# Autodesk Inventor assembly: Assembly X-Quad
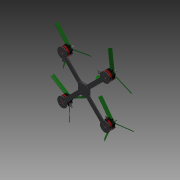
[picture p0: Inventor's stored thumbnail of the model, 180x180]
Saved by Autodesk Inventor 2015 (Build 190159000, 159)
## iProperties
Created: 2016-11-27
Part Number: Assembly X-Quad
Document SubType Name: Assembly
Designer: Hampus
Author: Hampus
## Documents named in this file (6)
- C:\Users\Hampus.Hampus-Dator\Desktop\Gymnasiearbete\Assembly X-Quad.iam
- C:\Users\Hampus.Hampus-Dator\Desktop\Gymnasiearbete\top.ipt
- C:\Users\Hampus.Hampus-Dator\Desktop\Gymnasiearbete\arm.ipt
- C:\Users\Hampus.Hampus-Dator\Desktop\Gymnasiearbete\botten.ipt
- D:\CAD3\Emax RS2205.ipt
- C:\Users\Hampus.Hampus-Dator\Desktop\Gymnasiearbete\DAL T5040.ipt
## Components (14 placed, 5 different names)
1. top:1 — Cylindrical:1, Rigid:1, Rigid:2, Cylindrical:2, Rotational:1
2. arm:1 — Rigid:2, Rotational:4
3. arm:2 — Cylindrical:1, Rotational:3
4. arm:3 — Cylindrical:2, Rotational:2
5. arm:4 — Rigid:1, Rigid:3
6. botten:1 — Rotational:1
7. Emax RS2205:1 — Rotational:4, Rigid:5
8. Emax RS2205:2 — Rigid:3, Rigid:4
9. Emax RS2205:3 — Rotational:3, Rigid:7
10. Emax RS2205:4 — Rotational:2, Rigid:6
11. DAL T5040:1 — Rigid:7
12. DAL T5040:2 — Rigid:6
13. DAL T5040:3 — Rigid:5
14. DAL T5040:4 — Rigid:4
## Relationships (13: WeldJoint 7, RevoluteJoint 4, CylindricalJoint 2)
- Cylindrical:1: top:1 ↔ arm:2
- Rigid:1 [WeldJoint]: top:1 ↔ arm:4
- Rigid:2 [WeldJoint]: top:1 ↔ arm:1
- Cylindrical:2: top:1 ↔ arm:3
- Rotational:1 [RevoluteJoint]: top:1 ↔ botten:1
- Rotational:2 [RevoluteJoint]: arm:3 ↔ Emax RS2205:4
- Rotational:3 [RevoluteJoint]: arm:2 ↔ Emax RS2205:3
- Rigid:3 [WeldJoint]: arm:4 ↔ Emax RS2205:2
- Rotational:4 [RevoluteJoint]: arm:1 ↔ Emax RS2205:1
- Rigid:4 [WeldJoint]: Emax RS2205:2 ↔ DAL T5040:4
- Rigid:5 [WeldJoint]: Emax RS2205:1 ↔ DAL T5040:3
- Rigid:6 [WeldJoint]: Emax RS2205:4 ↔ DAL T5040:2
- Rigid:7 [WeldJoint]: Emax RS2205:3 ↔ DAL T5040:1
